# Autodesk Inventor assembly: 組合1(更)
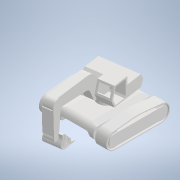
[picture p0: Inventor's stored thumbnail of the model, 180x180]
Saved by Autodesk Inventor 2020 (Build 240168000, 168)
## iProperties
Created: 2021-03-15
Part Number: 組合1(更)
Document SubType Name: Assembly
Designer: Sugar
Author: Sugar
## Documents named in this file (7)
- D:\諭\雷射切割\雷射切割-立體\組合1(更).iam
- D:\諭\雷射切割\雷射切割-立體\雷射切割5.ipt
- D:\諭\雷射切割\雷射切割-立體\雷射切割6.ipt
- D:\諭\雷射切割\雷射切割-立體\雷射切割1.ipt
- D:\諭\雷射切割\雷射切割-立體\雷射切割2.ipt
- D:\諭\雷射切割\雷射切割-立體\雷射切割3.ipt
- D:\諭\雷射切割\雷射切割-立體\雷射切割4.ipt
## Components (7 placed, 6 different names)
1. 雷射切割5:1 — 插入:1, 插入:2, 貼合:1, 貼合:2, 貼合:3, 貼合:7, 貼合:8
2. 雷射切割6:1 — 插入:1, 插入:2
3. 雷射切割6:2 — 貼合:1, 貼合:2, 貼合:3
4. 雷射切割1:1 — 貼合:5, 貼合:6, 貼合:8, 插入:3
5. 雷射切割2:1 — 插入:3, 插入:4, 角度:1
6. 雷射切割3:1 — 插入:4, 貼合:9, 貼合:10, 角度:1, 角度:2
7. 雷射切割4:1 — 貼合:9, 貼合:10, 角度:2
## Relationships (15: Mate 9, Insert 4, Angle 2)
- 插入:1 [Insert]: 雷射切割5:1 ↔ 雷射切割6:1
- 插入:2 [Insert]: 雷射切割5:1 ↔ 雷射切割6:1
- 貼合:1 [Mate]: 雷射切割5:1 ↔ 雷射切割6:2
- 貼合:2 [Mate]: 雷射切割5:1 ↔ 雷射切割6:2
- 貼合:3 [Mate]: 雷射切割5:1 ↔ 雷射切割6:2
- 貼合:5 [Mate]: 雷射切割1:1
- 貼合:6 [Mate]: 雷射切割1:1
- 貼合:7 [Mate]: 雷射切割5:1
- 貼合:8 [Mate]: 雷射切割5:1 ↔ 雷射切割1:1
- 插入:3 [Insert]: 雷射切割1:1 ↔ 雷射切割2:1
- 插入:4 [Insert]: 雷射切割2:1 ↔ 雷射切割3:1
- 貼合:9 [Mate]: 雷射切割3:1 ↔ 雷射切割4:1
- 貼合:10 [Mate]: 雷射切割3:1 ↔ 雷射切割4:1
- 角度:1 [Angle] (270 deg): 雷射切割2:1 ↔ 雷射切割3:1
- 角度:2 [Angle] (270 deg): 雷射切割3:1 ↔ 雷射切割4:1
